# Autodesk Inventor assembly: Combined Assembly
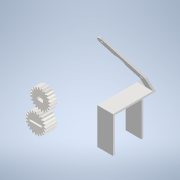
[picture p0: Inventor's stored thumbnail of the model, 180x180]
Saved by Autodesk Inventor 2021 (Build 250183000, 183)
## iProperties
Created: 2020-12-19
Part Number: Combined Assembly
Document SubType Name: Assembly
Designer: Ramsey
Author: Ramsey
## Documents named in this file (3)
- C:\Users\ramse\Documents\hackumass-blindcontrol\CAD\Combined Assembly.iam
- C:\Users\ramse\Documents\hackumass-blindcontrol\CAD\Gear Assembly.iam
- C:\Users\ramse\Documents\hackumass-blindcontrol\CAD\Motor Mount.ipt
## Components (2 placed, 2 different names)
1. Spur Gears:1 [sub-assembly] — Mate:1, Mate:2
2. Motor Mount:1
## Relationships (2: Mate 2)
- Mate:1: Spur Gears:1
- Mate:2: Spur Gears:1
